# Autodesk Inventor assembly: CrowsNestFinal-ver2-1111-2021
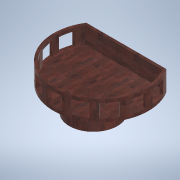
[picture p0: Inventor's stored thumbnail of the model, 180x180]
Saved by Autodesk Inventor 2021 (Build 250183000, 183)
## iProperties
Created: 2021-03-02
Part Number: CrowsNestFinal-ver2-1111-2021
Document SubType Name: Assembly
Designer: CMurray
Author: CMurray
## Documents named in this file (4)
- F:\PHRC CADD 2021\2021 Game Design Challenge\Crow's Nest\Assemblies\CrowsNestFinal-ver2-1111-2021.iam
- F:\PHRC CADD 2021\2021 Game Design Challenge\Crow's Nest\Parts\Nest-ver3-1111-2021.ipt
- F:\PHRC CADD 2021\2021 Game Design Challenge\Crow's Nest\Parts\NestTop-ver2-1111-2021.ipt
- F:\PHRC CADD 2021\2021 Game Design Challenge\Crow's Nest\Parts\NestPost-ver1-1111-2021.ipt
## Components (3 placed, 3 different names)
1. Nest-ver3-1111-2021:1 — Mate:1, Flush:1, Mate:2, Mate:3
2. NestTop-ver2-1111-2021:1 — Mate:1, Flush:1, Mate:2
3. NestPost-ver1-1111-2021:1 — Mate:3
## Relationships (4: Mate 3, Flush 1)
- Mate:1: Nest-ver3-1111-2021:1 ↔ NestTop-ver2-1111-2021:1
- Flush:1: Nest-ver3-1111-2021:1 ↔ NestTop-ver2-1111-2021:1
- Mate:2: Nest-ver3-1111-2021:1 ↔ NestTop-ver2-1111-2021:1
- Mate:3: Nest-ver3-1111-2021:1 ↔ NestPost-ver1-1111-2021:1
